# Autodesk Inventor assembly: 555
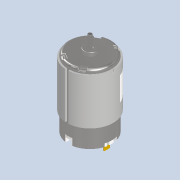
[picture p0: Inventor's stored thumbnail of the model, 180x180]
Saved by Autodesk Inventor 2021 (Build 250183000, 183)
## iProperties
Created: 2021-08-07
Part Number: 555
Document SubType Name: Assembly
Designer: Hagihara Yuya
Mass: 250 g
Surface Area: 278.556 cm^2
Volume: 20.0269 cm^3
Author: Hagihara Yuya
## Documents named in this file (9)
- C:\Users\Hagihara Yuya\Documents\GrabCAD\NHK2021\BasicParts\よく使う部品（萩原）\Motor\555\555.iam
- C:\Users\Hagihara Yuya\Documents\GrabCAD\NHK2021\BasicParts\よく使う部品（萩原）\Motor\555\555_Body.ipt
- C:\Users\Hagihara Yuya\Documents\GrabCAD\NHK2021\BasicParts\よく使う部品（萩原）\Motor\555\555_Outer.ipt
- C:\Users\Hagihara Yuya\Documents\GrabCAD\NHK2021\BasicParts\よく使う部品（萩原）\Motor\555\555_Cap.ipt
- C:\Users\Hagihara Yuya\Documents\GrabCAD\NHK2021\BasicParts\よく使う部品（萩原）\Motor\555\555_CapAccessory_1.ipt
- C:\Users\Hagihara Yuya\Documents\GrabCAD\NHK2021\BasicParts\よく使う部品（萩原）\Motor\555\555_CapAccessory_2.ipt
- C:\Users\Hagihara Yuya\Documents\GrabCAD\NHK2021\BasicParts\よく使う部品（萩原）\Motor\555\555_Terminal.ipt
- C:\Users\Hagihara Yuya\Documents\GrabCAD\NHK2021\BasicParts\よく使う部品（萩原）\Motor\555\555_CapAccessory_center.ipt
- C:\Users\Hagihara Yuya\Documents\GrabCAD\NHK2021\BasicParts\よく使う部品（萩原）\Motor\555\555_Shaft.ipt
## Components (11 placed, 8 different names)
1. 555_Body:1 — 回転:2, メイト:1, リジッド:1, メイト:3, メイト:5, フラッシュ:2, メイト:9
2. 555_Outer:1 — 回転:2, メイト:1
3. 555_Cap:1 — リジッド:1, メイト:2, フラッシュ:1, メイト:4, メイト:6, メイト:7, フラッシュ:3, メイト:8, メイト:10, 回転:3, 回転:4
4. 555_CapAccessory_1:1 — メイト:2, メイト:3, フラッシュ:1
5. 555_CapAccessory_1:2 — メイト:4, メイト:5, メイト:6
6. 555_CapAccessory_2:1 — メイト:7, フラッシュ:2, フラッシュ:3, メイト:11, フラッシュ:4, フラッシュ:5
7. 555_CapAccessory_2:2 — メイト:8, メイト:9, メイト:10, メイト:12, フラッシュ:6, フラッシュ:7
8. 555_Terminal:1 — メイト:11, フラッシュ:4, フラッシュ:5
9. 555_Terminal:2 — メイト:12, フラッシュ:6, フラッシュ:7
10. 555_CapAccessory_center:1 — 回転:3
11. 555_Shaft:1 — 回転:4
## Relationships (23: Mate 12, Flush 7, RevoluteJoint 3, WeldJoint 1)
- 回転:2 [RevoluteJoint] (3.3 mm): 555_Body:1 ↔ 555_Outer:1
- メイト:1 [Mate]: 555_Body:1 ↔ 555_Outer:1
- リジッド:1 [WeldJoint]: 555_Body:1 ↔ 555_Cap:1
- メイト:2 [Mate]: 555_Cap:1 ↔ 555_CapAccessory_1:1
- メイト:3 [Mate]: 555_Body:1 ↔ 555_CapAccessory_1:1
- フラッシュ:1 [Flush]: 555_Cap:1 ↔ 555_CapAccessory_1:1
- メイト:4 [Mate]: 555_Cap:1 ↔ 555_CapAccessory_1:2
- メイト:5 [Mate]: 555_Body:1 ↔ 555_CapAccessory_1:2
- メイト:6 [Mate]: 555_Cap:1 ↔ 555_CapAccessory_1:2
- メイト:7 [Mate]: 555_Cap:1 ↔ 555_CapAccessory_2:1
- フラッシュ:2 [Flush]: 555_Body:1 ↔ 555_CapAccessory_2:1
- フラッシュ:3 [Flush]: 555_Cap:1 ↔ 555_CapAccessory_2:1
- メイト:8 [Mate]: 555_Cap:1 ↔ 555_CapAccessory_2:2
- メイト:9 [Mate]: 555_Body:1 ↔ 555_CapAccessory_2:2
- メイト:10 [Mate]: 555_Cap:1 ↔ 555_CapAccessory_2:2
- メイト:11 [Mate]: 555_CapAccessory_2:1 ↔ 555_Terminal:1
- フラッシュ:4 [Flush]: 555_CapAccessory_2:1 ↔ 555_Terminal:1
- フラッシュ:5 [Flush]: 555_CapAccessory_2:1 ↔ 555_Terminal:1
- メイト:12 [Mate]: 555_CapAccessory_2:2 ↔ 555_Terminal:2
- フラッシュ:6 [Flush]: 555_CapAccessory_2:2 ↔ 555_Terminal:2
- フラッシュ:7 [Flush]: 555_CapAccessory_2:2 ↔ 555_Terminal:2
- 回転:3 [RevoluteJoint] (1 mm): 555_Cap:1 ↔ 555_CapAccessory_center:1
- 回転:4 [RevoluteJoint] (-10.7 mm): 555_Cap:1 ↔ 555_Shaft:1
